# Autodesk Inventor assembly: HS-7940TH Servo
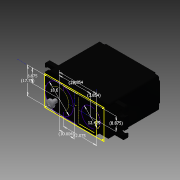
[picture p0: Inventor's stored thumbnail of the model, 180x180]
Saved by Autodesk Inventor 2015 (Build 190159000, 159)
## iProperties
Created: 2014-05-18
Part Number: HS-7940TH Servo
Document SubType Name: Assembly
Designer: seaha_000
Author: seaha_000
## Documents named in this file (7)
- C:\Users\Mosfet\Dropbox\_School\AimBot\HS-7940TH Servo.iam
- C:\Users\Mosfet\Dropbox\_School\AimBot\Imported Components\SW3dPS-Hitec Servo\Part7.ipt
- C:\Users\Mosfet\Dropbox\_School\AimBot\Imported Components\SW3dPS-Hitec Servo\Part9.ipt
- C:\Users\Mosfet\Dropbox\_School\AimBot\Imported Components\SW3dPS-Hitec Servo\Part11.ipt
- C:\Users\Mosfet\Dropbox\_School\AimBot\Imported Components\SW3dPS-Hitec Servo\Part13.ipt
- C:\Users\Mosfet\Dropbox\_School\AimBot\Imported Components\SW3dPS-Hitec Servo\Part15.ipt
- C:\Users\Mosfet\Dropbox\_School\AimBot\Imported Components\SW3dPS-Hitec Servo\Part27.ipt
## Components (6 placed, 6 different names)
1. Part7:1 — Mate:1, Mate:2, Mate:3, Mate:4, Mate:5, Mate:6, Mate:7, Mate:8, Mate:10
2. Part9:1 — Mate:5, Mate:6
3. Part11:1 — Mate:1, Mate:2
4. Part13:1 — Mate:3, Mate:4
5. Part15:1 — Mate:7, Mate:8
6. Part27:1 — Mate:10
## Relationships (9: Mate 9)
- Mate:1: Part7:1 ↔ Part11:1
- Mate:2: Part7:1 ↔ Part11:1
- Mate:3: Part7:1 ↔ Part13:1
- Mate:4: Part7:1 ↔ Part13:1
- Mate:5: Part7:1 ↔ Part9:1
- Mate:6: Part7:1 ↔ Part9:1
- Mate:7: Part7:1 ↔ Part15:1
- Mate:8: Part7:1 ↔ Part15:1
- Mate:10: Part7:1 ↔ Part27:1
